# Autodesk Inventor assembly: bed
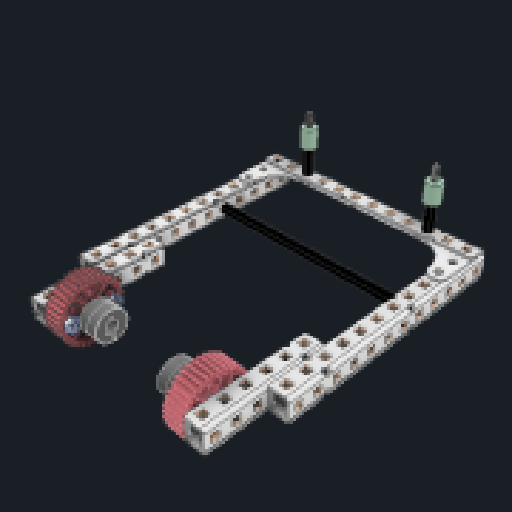
[picture p0: Inventor's stored thumbnail of the model, 512x512]
Saved by Autodesk Inventor 2024 (Build 280153000, 153)
## iProperties
Created: 2023-08-16
Part Number: bed
Document SubType Name: Assembly
Designer: avere
Author: avere
## Documents named in this file (13)
- C:\Users\Averey\Documents\vex\cad\scrap_v0.1\catapult\bed.iam
- C:\Users\Averey\Documents\vex\cad\scrap_v0.1\catapult\arm.iam
- C:\Users\Averey\Documents\vex\cad\scrap_v0.1\catapult\mirrored_parts\arm_MIR.iam
- C:\Users\Averey\Documents\vex\cad\VEX-CAD-Inventor-1.41\Structure\Angle\Aluminum 1x1\Alu Angle 1x1x12.ipt
- C:\Users\Averey\Documents\vex\cad\VEX-CAD-Inventor-1.41\Structure\Hardware\Rubber Link.ipt
- C:\Users\Averey\Documents\vex\cad\VEX-CAD-Inventor-1.41\Structure\Standoff\Standoff .75.ipt
- C:\Users\Averey\Documents\vex\cad\VEX-CAD-Inventor-1.41\Structure\Standoff\Standoff 5.00.ipt
- C:\Users\Averey\Documents\vex\cad\VEX-CAD-Inventor-1.41\Motion\Spacers\Washer Steel\SWasher .375 OD x .031250.ipt
- C:\Users\Averey\Documents\vex\cad\VEX-CAD-Inventor-1.41\Motion\Spacers\Washer Steel\SWasher .375 OD x .015625.ipt
- C:\Users\Averey\Documents\vex\cad\VEX-CAD-Inventor-1.41\Motion\Spacers\Washer Teflon\TWasher .375 OD x .04000.ipt
- D:\cad\VEX-CAD-Inventor-1.41\Structure\Standoff.ipt
- D:\cad\VEX-CAD-Inventor-1.41\Motion\Spacers\Washer Steel.ipt
- D:\cad\VEX-CAD-Inventor-1.41\Motion\Spacers\Washer Teflon.ipt
## Components (12 placed, 9 different names)
1. arm:1 [sub-assembly] — Insert:18, Insert:21, Insert:23, Mate:3
2. arm_MIR:1 [sub-assembly] — Mate:1, Insert:21, Insert:22, Mate:2
3. Alu Angle 1x1x12:1 — Insert:9, Insert:11, Insert:22, Mate:2, Insert:23, Mate:3
4. Alu Angle 1x1x12:2
5. Rubber Link:1 — Insert:8
6. Standoff .75:3 — Insert:8, Insert:9
7. Rubber Link:2
8. Standoff .75:4 — Insert:11
9. Standoff 5.00:5 — Insert:17, Mate:1
10. SWasher .375 OD x .031250:1 — Insert:16, Insert:17
11. SWasher .375 OD x .015625:2 — Insert:15, Insert:16
12. TWasher .375 OD x .04000:1 — Insert:15, Insert:18
## Relationships (14: Insert 11, Mate 3)
- Insert:8: Rubber Link:1 ↔ Standoff .75:3
- Insert:9: Alu Angle 1x1x12:1 ↔ Standoff .75:3
- [Insert]: Rubber Link:2 ↔ Standoff .75:4
- Insert:11: Alu Angle 1x1x12:1 ↔ Standoff .75:4
- Insert:15: SWasher .375 OD x .015625:2 ↔ TWasher .375 OD x .04000:1
- Insert:16: SWasher .375 OD x .031250:1 ↔ SWasher .375 OD x .015625:2
- Insert:17: Standoff 5.00:5 ↔ SWasher .375 OD x .031250:1
- Insert:18: arm:1 ↔ TWasher .375 OD x .04000:1
- Mate:1: arm_MIR:1 ↔ Standoff 5.00:5
- Insert:21 (129.3368 mm): arm:1 ↔ arm_MIR:1
- Insert:22: arm_MIR:1 ↔ Alu Angle 1x1x12:1
- Mate:2: arm_MIR:1 ↔ Alu Angle 1x1x12:1
- Insert:23: arm:1 ↔ Alu Angle 1x1x12:1
- Mate:3: arm:1 ↔ Alu Angle 1x1x12:1
## Named parameters: d11_d9 = 0 mm
